# Autodesk Inventor assembly: Alamak
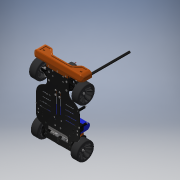
[picture p0: Inventor's stored thumbnail of the model, 180x180]
Saved by Autodesk Inventor 2019 (Build 230136000, 136)
## iProperties
Created: 2019-07-29
Part Number: Alamak
Material: Générique
Document SubType Name: Assembly
Designer: Sébastien DI MERCURIO
Author: Sébastien DI MERCURIO
## Documents named in this file (40)
- D:\Users\dimercur\Documents locaux\Travail\git\insa-nxpcup-1\meca\Inventor\Alamak.iam
- D:\Users\dimercur\Documents locaux\Travail\git\insa-nxpcup-1\meca\Inventor\Roulement.ipt
- D:\Users\dimercur\Documents locaux\Travail\git\insa-nxpcup-1\meca\Inventor\SupportMoteur.ipt
- D:\Users\dimercur\Documents locaux\Travail\git\insa-nxpcup-1\meca\Inventor\Base.ipt
- D:\Users\dimercur\Documents locaux\Travail\git\insa-nxpcup-1\meca\Inventor\Moteur.ipt
- D:\Users\dimercur\Documents locaux\Travail\git\insa-nxpcup-1\meca\Inventor\Plaque arriere.ipt
- D:\Users\dimercur\Documents locaux\Travail\git\insa-nxpcup-1\meca\Inventor\Content Center\fr-FR\ISO 7046-2 H\ISO 7046-2 H - M3x5 - 8.8 - H1.ipt
- D:\Users\dimercur\Documents locaux\Travail\git\insa-nxpcup-1\meca\Inventor\Pignon.ipt
- D:\Users\dimercur\Documents locaux\Travail\git\insa-nxpcup-1\meca\Inventor\PilierCentral.ipt
- D:\Users\dimercur\Documents locaux\Travail\git\insa-nxpcup-1\meca\Inventor\Content Center\fr-FR\ISO 7046-2 H\ISO 7046-2 H - M3x4 - 8.8 - H1.ipt
- D:\Users\dimercur\Documents locaux\Travail\git\insa-nxpcup-1\meca\Inventor\AxeArriere.ipt
- D:\Users\dimercur\Documents locaux\Travail\git\insa-nxpcup-1\meca\Inventor\Content Center\E4T-X-236-S-H-M-X.ipt
- D:\Users\dimercur\Documents locaux\Travail\git\insa-nxpcup-1\meca\Inventor\RoueDentée.ipt
- D:\Users\dimercur\Documents locaux\Travail\git\insa-nxpcup-1\meca\Inventor\Roue.ipt
- D:\Users\dimercur\Documents locaux\Travail\git\insa-nxpcup-1\meca\Inventor\Content Center\fr-FR\ANSI B18.16.3M(2)\ANSI B18.16.3M - Property Class 5 and 10 - Metric M3.5 x 0.6 Type de métal.ipt
- D:\Users\dimercur\Documents locaux\Travail\git\insa-nxpcup-1\meca\Inventor\EquerreBatterieGauche.ipt
- D:\Users\dimercur\Documents locaux\Travail\git\insa-nxpcup-1\meca\Inventor\EquerreBatterieDroite.ipt
- D:\Users\dimercur\Documents locaux\Travail\git\insa-nxpcup-1\meca\Inventor\SupportBatterie.ipt
- D:\Users\dimercur\Documents locaux\Travail\git\insa-nxpcup-1\meca\Inventor\Batterie.ipt
- D:\Users\dimercur\Documents locaux\Travail\git\insa-nxpcup-1\meca\Inventor\Content Center\fr-FR\NF EN ISO 7046-2 H\NF EN ISO 7046-2 H - M3x8 - 8.8 - H1.ipt
- D:\Users\dimercur\Documents locaux\Travail\git\insa-nxpcup-1\meca\Inventor\Content Center\fr-FR\ANSI B 18.2.4.1 M(1)\ANSI B 18.2.4.1 M - M2,5 x 0,45Style 1.ipt
- D:\Users\dimercur\Documents locaux\Travail\git\insa-nxpcup-1\meca\Inventor\EquerrePCBGauche.ipt
- D:\Users\dimercur\Documents locaux\Travail\git\insa-nxpcup-1\meca\Inventor\EquerrePCBDroite.ipt
- D:\Users\dimercur\Documents locaux\Travail\git\insa-nxpcup-1\meca\Inventor\Content Center\fr-FR\SS-ISO 7049 - F-H\ISO 7049 - ST2,2 x 13 - F - HSS-ISO.ipt
- D:\Users\dimercur\Documents locaux\Travail\git\insa-nxpcup-1\meca\Inventor\Content Center\fr-FR\SS-ISO 7049 - F-H\ISO 7049 - ST2,9 x 6,5 - F - HSS-ISO.ipt
- D:\Users\dimercur\Documents locaux\Travail\git\insa-nxpcup-1\meca\Inventor\SupportServo.ipt
- D:\Users\dimercur\Documents locaux\Travail\git\insa-nxpcup-1\meca\Inventor\Futaba S3003.ipt
- D:\Users\dimercur\Documents locaux\Travail\git\insa-nxpcup-1\meca\Inventor\Content Center\fr-FR\SS-ISO 7049 - F-H\ISO 7049 - ST4,2 x 9,5 - F - HSS-ISO.ipt
- D:\Users\dimercur\Documents locaux\Travail\git\insa-nxpcup-1\meca\Inventor\PieddeMat.ipt
- D:\Users\dimercur\Documents locaux\Travail\git\insa-nxpcup-1\meca\Inventor\Content Center\fr-FR\SFS EN ISO 7045 Z\EN ISO 7045 - M3 x 6 - 4.8 - Z(3).ipt
- D:\Users\dimercur\Documents locaux\Travail\git\insa-nxpcup-1\meca\Inventor\Content Center\fr-FR\ANSI B 18.2.4.1 M(1)\ANSI B 18.2.4.1 M - M3 x 0,5Style 1.ipt
- D:\Users\dimercur\Documents locaux\Travail\git\insa-nxpcup-1\meca\Inventor\Mat.ipt
- D:\Users\dimercur\Documents locaux\Travail\git\insa-nxpcup-1\meca\Inventor\Entretoise25mm.ipt
- D:\Users\dimercur\Documents locaux\Travail\git\insa-nxpcup-1\meca\Inventor\Content Center\fr-FR\SFS EN ISO 7045 Z\EN ISO 7045 - M3 x 8 - 4.8 - Z(3).ipt
- D:\Users\dimercur\Documents locaux\Travail\git\insa-nxpcup-1\meca\Inventor\Triangle.ipt
- D:\Users\dimercur\Documents locaux\Travail\git\insa-nxpcup-1\meca\Inventor\Content Center\fr-FR\NF EN ISO 7046-2 H\NF EN ISO 7046-2 H - M3.5x10 - 8.8 - H1.ipt
- D:\Users\dimercur\Documents locaux\Travail\git\insa-nxpcup-1\meca\Inventor\Fusée.ipt
- D:\Users\dimercur\Documents locaux\Travail\git\insa-nxpcup-1\meca\Inventor\PareChoc.ipt
- D:\Users\dimercur\Documents locaux\Travail\git\insa-nxpcup-1\meca\Inventor\Content Center\fr-FR\NF EN ISO 7046-2 H\NF EN ISO 7046-2 H - M3x12 - 8.8 - H1.ipt
- D:\Users\dimercur\Documents locaux\Travail\git\insa-nxpcup-1\meca\Inventor\GROVE-VL53L0X.ipt
## Components (124 placed, 39 different names)
1. Roulement:2 — Placage:1, Affleurement:1, Placage:37
2. Roulement:3 — Placage:2, Affleurement:2, Placage:36
3. SupportMoteur:1 — Placage:1, Affleurement:1, Placage:3, Placage:5, Placage:8, Placage:9, Tangente:2, Placage:13, Placage:74, Affleurement:9, Affleurement:10, Placage:77, Placage:79
4. SupportMoteur:2 — Placage:2, Affleurement:2, Placage:4, Placage:6, Placage:7, Placage:10, Tangente:1, Placage:11, Placage:12, Placage:75, Affleurement:11, Affleurement:12, Placage:82, Placage:83
5. Base:1 — Affleurement:3, Affleurement:4, Placage:3, Placage:4, Placage:5, Placage:6, Placage:7, Placage:8, Placage:18, Placage:19, Placage:21, Placage:22, Placage:23, Placage:24, Placage:27, Placage:30, Placage:31, Placage:54, Placage:56, Placage:57, Placage:58, Placage:59, Placage:60, Placage:61, Placage:62, Placage:63, Placage:67, Placage:68, Placage:69, Placage:70, Placage:71, Placage:72, Placage:73, Placage:87, Placage:88, Placage:89, Placage:93, Angle:3, Placage:94, Logement:23, Logement:24, Placage:96, Placage:98, Placage:110, Placage:111, Placage:112, Placage:115, Placage:116, Placage:117, Placage:118, Placage:119, Placage:120, Placage:121, Placage:122, Placage:123, Placage:124, Placage:125, Placage:126, Placage:127, Placage:128, Placage:137, Placage:138, Placage:139, Placage:144, Placage:166, Placage:169
6. Moteur:1 — Placage:9, Tangente:2, Placage:26, Affleurement:5
7. Moteur:2 — Placage:10, Tangente:1, Placage:25, Affleurement:6
8. Plaque arriere:1 — Placage:11, Placage:12, Placage:13, Placage:14, Placage:15, Placage:16, Placage:17, Placage:28, Placage:29, Placage:32, Placage:33
9. ISO 7046-2 H M3x5 - 8.8 - H1:1 — Placage:14
10. ISO 7046-2 H M3x5 - 8.8 - H1:2 — Placage:15
11. ISO 7046-2 H M3x5 - 8.8 - H1:3 — Placage:16
12. ISO 7046-2 H M3x5 - 8.8 - H1:4 — Placage:17
13. ISO 7046-2 H M3x5 - 8.8 - H1:5 — Placage:18
14. ISO 7046-2 H M3x5 - 8.8 - H1:6 — Placage:19
15. ISO 7046-2 H M3x5 - 8.8 - H1:7 — Placage:21
16. ISO 7046-2 H M3x5 - 8.8 - H1:8 — Placage:22
17. ISO 7046-2 H M3x5 - 8.8 - H1:9 — Placage:23
18. ISO 7046-2 H M3x5 - 8.8 - H1:10 — Placage:24
19. Pignon:1 — Placage:25, Affleurement:6, Placage:48
20. Pignon:2 — Placage:26, Affleurement:5, Placage:49
21. PilierCentral:1 — Placage:27, Placage:28, Placage:29, Placage:34, Affleurement:7, Affleurement:8, Placage:42, Placage:43
22. ISO 7046-2 H M3x4 - 8.8 - H1:1 — Placage:30
23. ISO 7046-2 H M3x5 - 8.8 - H1:11 — Placage:31
24. ISO 7046-2 H M3x5 - 8.8 - H1:12 — Placage:32
25. ISO 7046-2 H M3x5 - 8.8 - H1:13 — Placage:33
26. Roulement:4 — Placage:34, Affleurement:7, Placage:35, Placage:38
27. Roulement:5 — Placage:35, Affleurement:8, Placage:39
28. AxeArriere:1 — Placage:36, Placage:38, Placage:40, Placage:45, Placage:47, Placage:51
29. AxeArriere:2 — Placage:37, Placage:39, Placage:41, Placage:44, Placage:46, Placage:50
30. E4T-X-236-S-H-M-X:1 — Placage:41, Placage:42
31. E4T-X-236-S-H-M-X:2 — Placage:40, Placage:43
32. RoueDentée:1 — Placage:44, Placage:46, Placage:49, Placage:52, Angle:1
33. RoueDentée:2 — Placage:45, Placage:47, Placage:48, Placage:53, Angle:2
34. Roue:1 — Placage:50, Placage:52, Logement:1, Angle:1
35. Roue:2 — Placage:51, Placage:53, Logement:2, Angle:2
36. Ecrou hexagonal autofreiné - Acier Métrique Property Class 5 and 10 - Metric M3.5 x 0.6 Type de métal:1 — Logement:1
37. Ecrou hexagonal autofreiné - Acier Métrique Property Class 5 and 10 - Metric M3.5 x 0.6 Type de métal:2 — Logement:2
38. EquerreBatterieGauche:1 — Placage:54, Placage:56, Placage:57, Placage:64, Placage:65, Tangente:3, Logement:7, Logement:8, Placage:143
39. EquerreBatterieDroite:1 — Placage:58, Placage:59, Placage:60, Logement:9, Logement:10
40. SupportBatterie:1 — Placage:61, Placage:62, Placage:63, Logement:3, Logement:4, Logement:5, Logement:6
41. Batterie:1 — Placage:64, Placage:65, Tangente:3
42. NF EN ISO 7046-2 H M3x8 - 8.8 - H1:2 — Placage:67
43. NF EN ISO 7046-2 H M3x8 - 8.8 - H1:3 — Placage:68
44. NF EN ISO 7046-2 H M3x8 - 8.8 - H1:4 — Placage:69
45. NF EN ISO 7046-2 H M3x8 - 8.8 - H1:5 — Placage:70
46. NF EN ISO 7046-2 H M3x8 - 8.8 - H1:6 — Placage:71
47. NF EN ISO 7046-2 H M3x8 - 8.8 - H1:7 — Placage:72
48. NF EN ISO 7046-2 H M3x8 - 8.8 - H1:8 — Placage:73
49. Ecrou hexagonal Métrique M2,5 x 0,45:1 — Logement:3
50. Ecrou hexagonal Métrique M2,5 x 0,45:2 — Logement:4
51. Ecrou hexagonal Métrique M2,5 x 0,45:3 — Logement:5
52. Ecrou hexagonal Métrique M2,5 x 0,45:4 — Logement:6
53. Ecrou hexagonal Métrique M2,5 x 0,45:5 — Logement:7
54. Ecrou hexagonal Métrique M2,5 x 0,45:6 — Logement:8
55. Ecrou hexagonal Métrique M2,5 x 0,45:7 — Logement:9
56. Ecrou hexagonal Métrique M2,5 x 0,45:8 — Logement:10
57. EquerrePCBGauche:1 — Placage:74, Affleurement:9, Affleurement:10, Placage:76, Placage:78
58. EquerrePCBDroite:1 — Placage:75, Affleurement:11, Affleurement:12, Placage:80, Placage:81
59. SS ISO 7049 - F-H ST2,2 x 13 - F - H:1 — Placage:76, Placage:77
60. SS ISO 7049 - F-H ST2,2 x 13 - F - H:2 — Placage:78, Placage:79
61. SS ISO 7049 - F-H ST2,2 x 13 - F - H:3 — Placage:81, Placage:83
62. SS ISO 7049 - F-H ST2,2 x 13 - F - H:4 — Placage:80, Placage:82
63. SS ISO 7049 - F-H ST2,9 x 6,5 - F - H:1
64. SS ISO 7049 - F-H ST2,9 x 6,5 - F - H:2
65. SS ISO 7049 - F-H ST2,9 x 6,5 - F - H:3
66. SS ISO 7049 - F-H ST2,9 x 6,5 - F - H:4
67. SupportServo:1 — Placage:87, Placage:88, Placage:89, Placage:90, Placage:91, Placage:92, Logement:33, Logement:34, Logement:35, Logement:36
68. Futaba S3003:1 — Placage:90, Placage:91, Placage:92, Logement:15, Logement:16, Logement:17, Logement:18
69. SS ISO 7049 - F-H ST4,2 x 9,5 - F - H:1 — Logement:15
70. SS ISO 7049 - F-H ST4,2 x 9,5 - F - H:2 — Logement:16
71. SS ISO 7049 - F-H ST4,2 x 9,5 - F - H:3 — Logement:17
72. SS ISO 7049 - F-H ST4,2 x 9,5 - F - H:4 — Logement:18
73. PieddeMat:1 — Placage:93, Angle:3, Placage:94, Logement:19, Logement:20, Logement:21, Logement:22, Placage:99, Placage:100
74. SFS EN ISO 7045 Z M3 x 6 - 4.8 - Z:1 — Logement:19
75. SFS EN ISO 7045 Z M3 x 6 - 4.8 - Z:2 — Logement:20
76. SFS EN ISO 7045 Z M3 x 6 - 4.8 - Z:3 — Logement:21, Placage:97
77. SFS EN ISO 7045 Z M3 x 6 - 4.8 - Z:4 — Logement:22, Placage:95
78. Ecrou hexagonal Métrique M2,5 x 0,45:9 — Logement:23
79. Ecrou hexagonal Métrique M2,5 x 0,45:10 — Logement:24
80. Ecrou hexagonal Métrique M3 x 0,5:1 — Placage:95, Placage:96
81. Ecrou hexagonal Métrique M3 x 0,5:2 — Placage:97, Placage:98
82. Mat:1 — Placage:99, Placage:100
83. Entretoise25mm:1 — Logement:31, Placage:166, Placage:167
84. Entretoise25mm:2 — Logement:32, Placage:168
85. Entretoise25mm:3 — Placage:110, Logement:30, Placage:170
86. Entretoise25mm:4 — Placage:111, Placage:112, Logement:29, Placage:158, Placage:169
87. SFS EN ISO 7045 Z M3 x 8 - 4.8 - Z:1 — Placage:158
88. SFS EN ISO 7045 Z M3 x 8 - 4.8 - Z:2 — Placage:170
89. SFS EN ISO 7045 Z M3 x 8 - 4.8 - Z:3 — Placage:168
90. SFS EN ISO 7045 Z M3 x 8 - 4.8 - Z:4 — Placage:167
91. SFS EN ISO 7045 Z M3 x 8 - 4.8 - Z:5 — Logement:29
92. SFS EN ISO 7045 Z M3 x 8 - 4.8 - Z:6 — Logement:30
93. SFS EN ISO 7045 Z M3 x 8 - 4.8 - Z:7 — Logement:31
94. SFS EN ISO 7045 Z M3 x 8 - 4.8 - Z:8 — Logement:32
95. Triangle:1 — Placage:116, Placage:118, Placage:120, Placage:129, Placage:132
96. Triangle:2 — Placage:115, Placage:117, Placage:119, Placage:130, Placage:131
97. NF EN ISO 7046-2 H M3.5x10 - 8.8 - H1:1 — Placage:121
98. NF EN ISO 7046-2 H M3.5x10 - 8.8 - H1:2 — Placage:122
99. NF EN ISO 7046-2 H M3.5x10 - 8.8 - H1:3 — Placage:123
100. NF EN ISO 7046-2 H M3.5x10 - 8.8 - H1:4 — Placage:124
101. NF EN ISO 7046-2 H M3x8 - 8.8 - H1:9 — Placage:125
102. NF EN ISO 7046-2 H M3x8 - 8.8 - H1:10 — Placage:126
103. NF EN ISO 7046-2 H M3x8 - 8.8 - H1:11 — Placage:127
104. NF EN ISO 7046-2 H M3x8 - 8.8 - H1:12 — Placage:128
105. Ecrou hexagonal Métrique M2,5 x 0,45:11 — Logement:33
106. Ecrou hexagonal Métrique M2,5 x 0,45:12 — Logement:34
107. Ecrou hexagonal Métrique M2,5 x 0,45:13 — Logement:35
108. Ecrou hexagonal Métrique M2,5 x 0,45:14 — Logement:36
109. Fusée:1 — Placage:129, Placage:132, Placage:134, Placage:136, Angle:6
110. Fusée:2 — Placage:130, Placage:131, Placage:133, Placage:135, Angle:6
111. Roue:3 — Placage:133, Placage:135, Logement:38
112. Roue:4 — Placage:134, Placage:136, Logement:37
113. Ecrou hexagonal autofreiné - Acier Métrique Property Class 5 and 10 - Metric M3.5 x 0.6 Type de métal:3 — Logement:37
114. Ecrou hexagonal autofreiné - Acier Métrique Property Class 5 and 10 - Metric M3.5 x 0.6 Type de métal:4 — Logement:38
115. PareChoc:1 — Placage:137, Placage:138, Placage:139, Placage:140, Placage:141, Placage:142, Logement:39, Logement:40, Logement:41, Placage:171, Placage:172, Placage:173, Placage:174, Placage:175, Placage:176
116. NF EN ISO 7046-2 H M3x12 - 8.8 - H1:1 — Placage:140
117. NF EN ISO 7046-2 H M3x12 - 8.8 - H1:2 — Placage:141
118. NF EN ISO 7046-2 H M3x12 - 8.8 - H1:3 — Placage:142
119. Ecrou hexagonal Métrique M2,5 x 0,45:15 — Logement:39
120. Ecrou hexagonal Métrique M2,5 x 0,45:16 — Logement:40
121. Ecrou hexagonal Métrique M2,5 x 0,45:17 — Logement:41
122. NF EN ISO 7046-2 H M3x8 - 8.8 - H1:13 — Placage:143, Placage:144
123. GROVE-VL53L0X:1 — Placage:172, Placage:175, Placage:176
124. GROVE-VL53L0X:2 — Placage:171, Placage:173, Placage:174
## Relationships (191: Mate 139, Insert 33, Flush 12, Angle 4, Tangent 3)
- Placage:1 [Mate]: Roulement:2 ↔ SupportMoteur:1
- Placage:2 [Mate]: Roulement:3 ↔ SupportMoteur:2
- Affleurement:1 [Flush]: Roulement:2 ↔ SupportMoteur:1
- Affleurement:2 [Flush]: Roulement:3 ↔ SupportMoteur:2
- Affleurement:3 [Flush]: Base:1
- Affleurement:4 [Flush]: Base:1
- Placage:3 [Mate]: SupportMoteur:1 ↔ Base:1
- Placage:4 [Mate]: SupportMoteur:2 ↔ Base:1
- Placage:5 [Mate]: SupportMoteur:1 ↔ Base:1
- Placage:6 [Mate]: SupportMoteur:2 ↔ Base:1
- Placage:7 [Mate]: SupportMoteur:2 ↔ Base:1
- Placage:8 [Mate]: SupportMoteur:1 ↔ Base:1
- Placage:9 [Mate]: SupportMoteur:1 ↔ Moteur:1
- Placage:10 [Mate]: SupportMoteur:2 ↔ Moteur:2
- Tangente:1: SupportMoteur:2 ↔ Moteur:2
- Tangente:2: SupportMoteur:1 ↔ Moteur:1
- Placage:11 [Mate]: SupportMoteur:2 ↔ Plaque arriere:1
- Placage:12 [Mate]: SupportMoteur:2 ↔ Plaque arriere:1
- Placage:13 [Mate]: SupportMoteur:1 ↔ Plaque arriere:1
- Placage:14 [Mate]: Plaque arriere:1 ↔ ISO 7046-2 H M3x5 - 8.8 - H1:1
- Placage:15 [Mate]: Plaque arriere:1 ↔ ISO 7046-2 H M3x5 - 8.8 - H1:2
- Placage:16 [Mate]: Plaque arriere:1 ↔ ISO 7046-2 H M3x5 - 8.8 - H1:3
- Placage:17 [Mate]: Plaque arriere:1 ↔ ISO 7046-2 H M3x5 - 8.8 - H1:4
- Placage:18 [Mate]: Base:1 ↔ ISO 7046-2 H M3x5 - 8.8 - H1:5
- Placage:19 [Mate]: Base:1 ↔ ISO 7046-2 H M3x5 - 8.8 - H1:6
- Placage:21 [Mate]: Base:1 ↔ ISO 7046-2 H M3x5 - 8.8 - H1:7
- Placage:22 [Mate]: Base:1 ↔ ISO 7046-2 H M3x5 - 8.8 - H1:8
- Placage:23 [Mate]: Base:1 ↔ ISO 7046-2 H M3x5 - 8.8 - H1:9
- Placage:24 [Mate]: Base:1 ↔ ISO 7046-2 H M3x5 - 8.8 - H1:10
- Placage:25 [Mate]: Moteur:2 ↔ Pignon:1
- Placage:26 [Mate]: Moteur:1 ↔ Pignon:2
- Affleurement:5 [Flush] (-3 mm): Moteur:1 ↔ Pignon:2
- Affleurement:6 [Flush] (3 mm): Moteur:2 ↔ Pignon:1
- Placage:27 [Mate]: Base:1 ↔ PilierCentral:1
- Placage:28 [Mate]: Plaque arriere:1 ↔ PilierCentral:1
- Placage:29 [Mate]: Plaque arriere:1 ↔ PilierCentral:1
- Placage:30 [Mate]: Base:1 ↔ ISO 7046-2 H M3x4 - 8.8 - H1:1
- Placage:31 [Mate]: Base:1 ↔ ISO 7046-2 H M3x5 - 8.8 - H1:11
- Placage:32 [Mate]: Plaque arriere:1 ↔ ISO 7046-2 H M3x5 - 8.8 - H1:12
- Placage:33 [Mate]: Plaque arriere:1 ↔ ISO 7046-2 H M3x5 - 8.8 - H1:13
- Placage:34 [Mate]: PilierCentral:1 ↔ Roulement:4
- Affleurement:7 [Flush]: PilierCentral:1 ↔ Roulement:4
- Placage:35 [Mate]: Roulement:4 ↔ Roulement:5
- Affleurement:8 [Flush]: PilierCentral:1 ↔ Roulement:5
- Placage:36 [Mate]: Roulement:3 ↔ AxeArriere:1
- Placage:37 [Mate]: Roulement:2 ↔ AxeArriere:2
- Placage:38 [Mate]: Roulement:4 ↔ AxeArriere:1
- Placage:39 [Mate]: Roulement:5 ↔ AxeArriere:2
- Placage:40 [Mate]: AxeArriere:1 ↔ E4T-X-236-S-H-M-X:2
- Placage:41 [Mate]: AxeArriere:2 ↔ E4T-X-236-S-H-M-X:1
- Placage:42 [Mate]: PilierCentral:1 ↔ E4T-X-236-S-H-M-X:1
- Placage:43 [Mate]: PilierCentral:1 ↔ E4T-X-236-S-H-M-X:2
- Placage:44 [Mate]: AxeArriere:2 ↔ RoueDentée:1
- Placage:45 [Mate]: AxeArriere:1 ↔ RoueDentée:2
- Placage:46 [Mate]: AxeArriere:2 ↔ RoueDentée:1
- Placage:47 [Mate]: AxeArriere:1 ↔ RoueDentée:2
- Placage:48 [Mate]: Pignon:1 ↔ RoueDentée:2
- Placage:49 [Mate]: Pignon:2 ↔ RoueDentée:1
- Placage:50 [Mate]: AxeArriere:2 ↔ Roue:1
- Placage:51 [Mate]: AxeArriere:1 ↔ Roue:2
- Placage:52 [Mate]: RoueDentée:1 ↔ Roue:1
- Placage:53 [Mate]: RoueDentée:2 ↔ Roue:2
- Logement:1 [Insert]: Roue:1 ↔ Ecrou hexagonal autofreiné - Acier Métrique Property Class 5 and 10 - Metric M3.5 x 0.6 Type de métal:1
- Logement:2 [Insert]: Roue:2 ↔ Ecrou hexagonal autofreiné - Acier Métrique Property Class 5 and 10 - Metric M3.5 x 0.6 Type de métal:2
- Angle:1 (0 deg): RoueDentée:1 ↔ Roue:1
- Angle:2 (0 deg): RoueDentée:2 ↔ Roue:2
- Placage:54 [Mate]: Base:1 ↔ EquerreBatterieGauche:1
- Placage:56 [Mate]: Base:1 ↔ EquerreBatterieGauche:1
- Placage:57 [Mate]: Base:1 ↔ EquerreBatterieGauche:1
- Placage:58 [Mate]: Base:1 ↔ EquerreBatterieDroite:1
- Placage:59 [Mate]: Base:1 ↔ EquerreBatterieDroite:1
- Placage:60 [Mate]: Base:1 ↔ EquerreBatterieDroite:1
- Placage:61 [Mate]: Base:1 ↔ SupportBatterie:1
- Placage:62 [Mate]: Base:1 ↔ SupportBatterie:1
- Placage:63 [Mate]: Base:1 ↔ SupportBatterie:1
- Placage:64 [Mate]: EquerreBatterieGauche:1 ↔ Batterie:1
- Placage:65 [Mate]: EquerreBatterieGauche:1 ↔ Batterie:1
- Tangente:3: EquerreBatterieGauche:1 ↔ Batterie:1
- Placage:67 [Mate]: Base:1 ↔ NF EN ISO 7046-2 H M3x8 - 8.8 - H1:2
- Placage:68 [Mate]: Base:1 ↔ NF EN ISO 7046-2 H M3x8 - 8.8 - H1:3
- Placage:69 [Mate]: Base:1 ↔ NF EN ISO 7046-2 H M3x8 - 8.8 - H1:4
- Placage:70 [Mate]: Base:1 ↔ NF EN ISO 7046-2 H M3x8 - 8.8 - H1:5
- Placage:71 [Mate]: Base:1 ↔ NF EN ISO 7046-2 H M3x8 - 8.8 - H1:6
- Placage:72 [Mate]: Base:1 ↔ NF EN ISO 7046-2 H M3x8 - 8.8 - H1:7
- Placage:73 [Mate]: Base:1 ↔ NF EN ISO 7046-2 H M3x8 - 8.8 - H1:8
- Logement:3 [Insert]: SupportBatterie:1 ↔ Ecrou hexagonal Métrique M2,5 x 0,45:1
- Logement:4 [Insert]: SupportBatterie:1 ↔ Ecrou hexagonal Métrique M2,5 x 0,45:2
- Logement:5 [Insert]: SupportBatterie:1 ↔ Ecrou hexagonal Métrique M2,5 x 0,45:3
- Logement:6 [Insert]: SupportBatterie:1 ↔ Ecrou hexagonal Métrique M2,5 x 0,45:4
- Logement:7 [Insert]: EquerreBatterieGauche:1 ↔ Ecrou hexagonal Métrique M2,5 x 0,45:5
- Logement:8 [Insert]: EquerreBatterieGauche:1 ↔ Ecrou hexagonal Métrique M2,5 x 0,45:6
- Logement:9 [Insert]: EquerreBatterieDroite:1 ↔ Ecrou hexagonal Métrique M2,5 x 0,45:7
- Logement:10 [Insert]: EquerreBatterieDroite:1 ↔ Ecrou hexagonal Métrique M2,5 x 0,45:8
- Placage:74 [Mate]: SupportMoteur:1 ↔ EquerrePCBGauche:1
- Affleurement:9 [Flush] (-3 mm): SupportMoteur:1 ↔ EquerrePCBGauche:1
- Affleurement:10 [Flush] (0.5 mm): SupportMoteur:1 ↔ EquerrePCBGauche:1
- Placage:75 [Mate]: SupportMoteur:2 ↔ EquerrePCBDroite:1
- Affleurement:11 [Flush] (0.5 mm): SupportMoteur:2 ↔ EquerrePCBDroite:1
- Affleurement:12 [Flush] (-3 mm): SupportMoteur:2 ↔ EquerrePCBDroite:1
- Placage:76 [Mate]: EquerrePCBGauche:1 ↔ SS ISO 7049 - F-H ST2,2 x 13 - F - H:1
- Placage:77 [Mate]: SupportMoteur:1 ↔ SS ISO 7049 - F-H ST2,2 x 13 - F - H:1
- Placage:78 [Mate]: EquerrePCBGauche:1 ↔ SS ISO 7049 - F-H ST2,2 x 13 - F - H:2
- Placage:79 [Mate]: SupportMoteur:1 ↔ SS ISO 7049 - F-H ST2,2 x 13 - F - H:2
- Placage:80 [Mate]: EquerrePCBDroite:1 ↔ SS ISO 7049 - F-H ST2,2 x 13 - F - H:4
- Placage:81 [Mate]: EquerrePCBDroite:1 ↔ SS ISO 7049 - F-H ST2,2 x 13 - F - H:3
- Placage:82 [Mate]: SupportMoteur:2 ↔ SS ISO 7049 - F-H ST2,2 x 13 - F - H:4
- Placage:83 [Mate]: SupportMoteur:2 ↔ SS ISO 7049 - F-H ST2,2 x 13 - F - H:3
- Placage:87 [Mate]: Base:1 ↔ SupportServo:1
- Placage:88 [Mate]: Base:1 ↔ SupportServo:1
- Placage:89 [Mate]: Base:1 ↔ SupportServo:1
- Placage:90 [Mate]: SupportServo:1 ↔ Futaba S3003:1
- Placage:91 [Mate]: SupportServo:1 ↔ Futaba S3003:1
- Placage:92 [Mate]: SupportServo:1 ↔ Futaba S3003:1
- Logement:15 [Insert]: Futaba S3003:1 ↔ SS ISO 7049 - F-H ST4,2 x 9,5 - F - H:1
- Logement:16 [Insert]: Futaba S3003:1 ↔ SS ISO 7049 - F-H ST4,2 x 9,5 - F - H:2
- Logement:17 [Insert]: Futaba S3003:1 ↔ SS ISO 7049 - F-H ST4,2 x 9,5 - F - H:3
- Logement:18 [Insert]: Futaba S3003:1 ↔ SS ISO 7049 - F-H ST4,2 x 9,5 - F - H:4
- Placage:93 [Mate]: Base:1 ↔ PieddeMat:1
- Angle:3 (0 deg): Base:1 ↔ PieddeMat:1
- Placage:94 [Mate]: Base:1 ↔ PieddeMat:1
- Logement:19 [Insert]: PieddeMat:1 ↔ SFS EN ISO 7045 Z M3 x 6 - 4.8 - Z:1
- Logement:20 [Insert]: PieddeMat:1 ↔ SFS EN ISO 7045 Z M3 x 6 - 4.8 - Z:2
- Logement:21 [Insert]: PieddeMat:1 ↔ SFS EN ISO 7045 Z M3 x 6 - 4.8 - Z:3
- Logement:22 [Insert]: PieddeMat:1 ↔ SFS EN ISO 7045 Z M3 x 6 - 4.8 - Z:4
- Logement:23 [Insert]: Base:1 ↔ Ecrou hexagonal Métrique M2,5 x 0,45:9
- Logement:24 [Insert]: Base:1 ↔ Ecrou hexagonal Métrique M2,5 x 0,45:10
- Placage:95 [Mate]: SFS EN ISO 7045 Z M3 x 6 - 4.8 - Z:4 ↔ Ecrou hexagonal Métrique M3 x 0,5:1
- Placage:96 [Mate]: Base:1 ↔ Ecrou hexagonal Métrique M3 x 0,5:1
- Placage:97 [Mate]: SFS EN ISO 7045 Z M3 x 6 - 4.8 - Z:3 ↔ Ecrou hexagonal Métrique M3 x 0,5:2
- Placage:98 [Mate]: Base:1 ↔ Ecrou hexagonal Métrique M3 x 0,5:2
- Placage:99 [Mate]: PieddeMat:1 ↔ Mat:1
- Placage:100 [Mate] (15 mm): PieddeMat:1 ↔ Mat:1
- Placage:110 [Mate]: Base:1 ↔ Entretoise25mm:3
- Placage:111 [Mate] (15 mm): Base:1 ↔ Entretoise25mm:4
- Placage:112 [Mate] (1.5 mm): Base:1 ↔ Entretoise25mm:4
- Logement:29 [Insert]: Entretoise25mm:4 ↔ SFS EN ISO 7045 Z M3 x 8 - 4.8 - Z:5
- Logement:30 [Insert]: Entretoise25mm:3 ↔ SFS EN ISO 7045 Z M3 x 8 - 4.8 - Z:6
- Logement:31 [Insert]: Entretoise25mm:1 ↔ SFS EN ISO 7045 Z M3 x 8 - 4.8 - Z:7
- Logement:32 [Insert]: Entretoise25mm:2 ↔ SFS EN ISO 7045 Z M3 x 8 - 4.8 - Z:8
- Placage:115 [Mate]: Base:1 ↔ Triangle:2
- Placage:116 [Mate]: Base:1 ↔ Triangle:1
- Placage:117 [Mate]: Base:1 ↔ Triangle:2
- Placage:118 [Mate]: Base:1 ↔ Triangle:1
- Placage:119 [Mate]: Base:1 ↔ Triangle:2
- Placage:120 [Mate]: Base:1 ↔ Triangle:1
- Placage:121 [Mate]: Base:1 ↔ NF EN ISO 7046-2 H M3.5x10 - 8.8 - H1:1
- Placage:122 [Mate]: Base:1 ↔ NF EN ISO 7046-2 H M3.5x10 - 8.8 - H1:2
- Placage:123 [Mate]: Base:1 ↔ NF EN ISO 7046-2 H M3.5x10 - 8.8 - H1:3
- Placage:124 [Mate]: Base:1 ↔ NF EN ISO 7046-2 H M3.5x10 - 8.8 - H1:4
- Placage:125 [Mate]: Base:1 ↔ NF EN ISO 7046-2 H M3x8 - 8.8 - H1:9
- Placage:126 [Mate]: Base:1 ↔ NF EN ISO 7046-2 H M3x8 - 8.8 - H1:10
- Placage:127 [Mate]: Base:1 ↔ NF EN ISO 7046-2 H M3x8 - 8.8 - H1:11
- Placage:128 [Mate]: Base:1 ↔ NF EN ISO 7046-2 H M3x8 - 8.8 - H1:12
- Logement:33 [Insert]: SupportServo:1 ↔ Ecrou hexagonal Métrique M2,5 x 0,45:11
- Logement:34 [Insert]: SupportServo:1 ↔ Ecrou hexagonal Métrique M2,5 x 0,45:12
- Logement:35 [Insert]: SupportServo:1 ↔ Ecrou hexagonal Métrique M2,5 x 0,45:13
- Logement:36 [Insert]: SupportServo:1 ↔ Ecrou hexagonal Métrique M2,5 x 0,45:14
- Placage:129 [Mate]: Triangle:1 ↔ Fusée:1
- Placage:130 [Mate]: Triangle:2 ↔ Fusée:2
- Placage:131 [Mate]: Triangle:2 ↔ Fusée:2
- Placage:132 [Mate]: Triangle:1 ↔ Fusée:1
- Placage:133 [Mate]: Fusée:2 ↔ Roue:3
- Placage:134 [Mate]: Fusée:1 ↔ Roue:4
- Placage:135 [Mate]: Fusée:2 ↔ Roue:3
- Placage:136 [Mate]: Fusée:1 ↔ Roue:4
- Logement:37 [Insert]: Roue:4 ↔ Ecrou hexagonal autofreiné - Acier Métrique Property Class 5 and 10 - Metric M3.5 x 0.6 Type de métal:3
- Logement:38 [Insert]: Roue:3 ↔ Ecrou hexagonal autofreiné - Acier Métrique Property Class 5 and 10 - Metric M3.5 x 0.6 Type de métal:4
- Angle:6 (0 deg): Fusée:1 ↔ Fusée:2
- Placage:137 [Mate]: Base:1 ↔ PareChoc:1
- Placage:138 [Mate]: Base:1 ↔ PareChoc:1
- Placage:139 [Mate]: Base:1 ↔ PareChoc:1
- Placage:140 [Mate]: PareChoc:1 ↔ NF EN ISO 7046-2 H M3x12 - 8.8 - H1:1
- Placage:141 [Mate]: PareChoc:1 ↔ NF EN ISO 7046-2 H M3x12 - 8.8 - H1:2
- Placage:142 [Mate]: PareChoc:1 ↔ NF EN ISO 7046-2 H M3x12 - 8.8 - H1:3
- Logement:39 [Insert]: PareChoc:1 ↔ Ecrou hexagonal Métrique M2,5 x 0,45:15
- Logement:40 [Insert]: PareChoc:1 ↔ Ecrou hexagonal Métrique M2,5 x 0,45:16
- Logement:41 [Insert]: PareChoc:1 ↔ Ecrou hexagonal Métrique M2,5 x 0,45:17
- Placage:143 [Mate]: EquerreBatterieGauche:1 ↔ NF EN ISO 7046-2 H M3x8 - 8.8 - H1:13
- Placage:144 [Mate]: Base:1 ↔ NF EN ISO 7046-2 H M3x8 - 8.8 - H1:13
- Placage:158 [Mate]: Entretoise25mm:4 ↔ SFS EN ISO 7045 Z M3 x 8 - 4.8 - Z:1
- Placage:166 [Mate]: Base:1 ↔ Entretoise25mm:1
- Placage:167 [Mate]: Entretoise25mm:1 ↔ SFS EN ISO 7045 Z M3 x 8 - 4.8 - Z:4
- Placage:168 [Mate]: Entretoise25mm:2 ↔ SFS EN ISO 7045 Z M3 x 8 - 4.8 - Z:3
- Placage:169 [Mate]: Base:1 ↔ Entretoise25mm:4
- Placage:170 [Mate]: Entretoise25mm:3 ↔ SFS EN ISO 7045 Z M3 x 8 - 4.8 - Z:2
- Placage:171 [Mate]: PareChoc:1 ↔ GROVE-VL53L0X:2
- Placage:172 [Mate]: PareChoc:1 ↔ GROVE-VL53L0X:1
- Placage:173 [Mate]: PareChoc:1 ↔ GROVE-VL53L0X:2
- Placage:174 [Mate]: PareChoc:1 ↔ GROVE-VL53L0X:2
- Placage:175 [Mate]: PareChoc:1 ↔ GROVE-VL53L0X:1
- Placage:176 [Mate]: PareChoc:1 ↔ GROVE-VL53L0X:1
